# Autodesk Inventor assembly: 240614_체인2
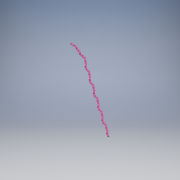
[picture p0: Inventor's stored thumbnail of the model, 180x180]
Saved by Autodesk Inventor 2016 (Build 200138000, 138)
## iProperties
Created: 2024-06-14
Part Number: 240614_체인2
Material: 일반
Document SubType Name: Assembly
Designer: pc
Author: pc
## Documents named in this file (2)
- D:\CAD_HCH\240614\240614_체인2.iam
- D:\CAD_HCH\240614\240614_체인.iam
## Components (7 placed, 1 different names)
1. 240614_체인:1 [sub-assembly] — 메이트:13, 메이트:14
2. 240614_체인:2 [sub-assembly] — 메이트:13, 메이트:14, 메이트:15, 메이트:16
3. 240614_체인:3 [sub-assembly] — 메이트:5, 메이트:6, 메이트:15, 메이트:16
4. 240614_체인:4 [sub-assembly] — 메이트:5, 메이트:6, 메이트:7, 메이트:8
5. 240614_체인:5 [sub-assembly] — 메이트:7, 메이트:8, 메이트:9, 메이트:10
6. 240614_체인:6 [sub-assembly] — 메이트:9, 메이트:10, 메이트:11, 메이트:12
7. 240614_체인:7 [sub-assembly] — 메이트:11, 메이트:12
## Relationships (12: Mate 12)
- 메이트:5 [Mate]: 240614_체인:3 ↔ 240614_체인:4
- 메이트:6 [Mate]: 240614_체인:3 ↔ 240614_체인:4
- 메이트:7 [Mate]: 240614_체인:4 ↔ 240614_체인:5
- 메이트:8 [Mate]: 240614_체인:4 ↔ 240614_체인:5
- 메이트:9 [Mate]: 240614_체인:5 ↔ 240614_체인:6
- 메이트:10 [Mate]: 240614_체인:5 ↔ 240614_체인:6
- 메이트:11 [Mate]: 240614_체인:6 ↔ 240614_체인:7
- 메이트:12 [Mate]: 240614_체인:6 ↔ 240614_체인:7
- 메이트:13 [Mate]: 240614_체인:1 ↔ 240614_체인:2
- 메이트:14 [Mate]: 240614_체인:1 ↔ 240614_체인:2
- 메이트:15 [Mate]: 240614_체인:2 ↔ 240614_체인:3
- 메이트:16 [Mate]: 240614_체인:2 ↔ 240614_체인:3
